# Autodesk Inventor assembly: 二号螺丝+防滑
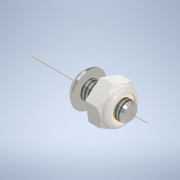
[picture p0: Inventor's stored thumbnail of the model, 180x180]
Saved by Autodesk Inventor 2020 (Build 240168000, 168)
## iProperties
Created: 2019-06-01
Part Number: 二号螺丝+防滑
Document SubType Name: Assembly
Designer: aresp
Author: aresp
## Documents named in this file (3)
- D:\vault\ncrCadLib\二号螺丝+防滑.iam
- D:\vault\ncrCadLib\螺丝螺帽\Screw 8-32 x 0.375'' 二号.ipt
- D:\vault\ncrCadLib\螺丝螺帽\防滑螺帽.ipt
## Components (2 placed, 2 different names)
1. Screw 8-32 x 0.375'' 二号:1 — 配合:1, 配合:2
2. 防滑螺帽:1 — 配合:1, 配合:2
## Relationships (2: Mate 2)
- 配合:1 [Mate]: Screw 8-32 x 0.375'' 二号:1 ↔ 防滑螺帽:1
- 配合:2 [Mate] (3.1496 mm): Screw 8-32 x 0.375'' 二号:1 ↔ 防滑螺帽:1
## Named parameters: 间隔距离 = 3.1496 mm
